# Autodesk Inventor assembly: держалка_мозговорота
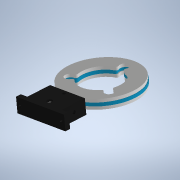
[picture p0: Inventor's stored thumbnail of the model, 180x180]
Saved by Autodesk Inventor 2021.1 (Build 251245010, 245A)
## iProperties
Created: 2022-11-16
Part Number: держалка_мозговорота
Document SubType Name: Assembly
Designer: zmoze
Author: zmoze
## Documents named in this file (5)
- C:\Users\zmoze\OneDrive\Рабочий стол\GrabCAD\Smile_2022-2023\держалка_мозговорота.iam
- C:\Users\zmoze\OneDrive\Рабочий стол\GrabCAD\Smile_2022-2023\Деталь1_мозговорот.ipt
- C:\Users\zmoze\OneDrive\Рабочий стол\GrabCAD\Smile_2022-2023\Деталь2_мозговорот.ipt
- C:\Users\zmoze\OneDrive\Рабочий стол\GrabCAD\Smile_2022-2023\Деталь3_мозговорот.ipt
- C:\Users\zmoze\OneDrive\Рабочий стол\GrabCAD\Smile_2022-2023\стаканчик_мозговорот.ipt
## Components (4 placed, 4 different names)
1. Деталь1_мозговорот:1 — Совмещение:1, Совмещение:4, Совмещение:8
2. Деталь2_мозговорот:1 — Совмещение:1, Совмещение:2, Совмещение:3, Совмещение:4
3. Деталь3_мозговорот:1 — Совмещение:2, Совмещение:3, Совмещение:5, Совмещение:6, Совмещение:7
4. стаканчик_мозговорот:1 — Совмещение:5, Совмещение:6, Совмещение:7, Совмещение:8
## Relationships (8: Mate 8)
- Совмещение:1 [Mate]: Деталь1_мозговорот:1 ↔ Деталь2_мозговорот:1
- Совмещение:2 [Mate]: Деталь2_мозговорот:1 ↔ Деталь3_мозговорот:1
- Совмещение:3 [Mate]: Деталь2_мозговорот:1 ↔ Деталь3_мозговорот:1
- Совмещение:4 [Mate]: Деталь1_мозговорот:1 ↔ Деталь2_мозговорот:1
- Совмещение:5 [Mate]: Деталь3_мозговорот:1 ↔ стаканчик_мозговорот:1
- Совмещение:6 [Mate]: Деталь3_мозговорот:1 ↔ стаканчик_мозговорот:1
- Совмещение:7 [Mate]: Деталь3_мозговорот:1 ↔ стаканчик_мозговорот:1
- Совмещение:8 [Mate]: Деталь1_мозговорот:1 ↔ стаканчик_мозговорот:1
